# Autodesk Inventor assembly: CL3-100
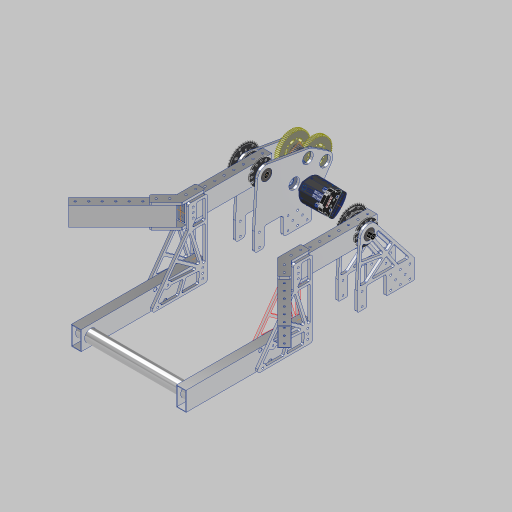
[picture p0: Inventor's stored thumbnail of the model, 512x512]
Saved by Autodesk Inventor 2023.5 (Build 275446000, 446)
## iProperties
Created: 2025-01-28
Part Number: CL3-100
Document SubType Name: Assembly
Designer: slick
Mass: 5966.39 g
Surface Area: 14199.1 cm^2
Volume: 2256.64 cm^3
Density: 2.64392 g/cm^3
Author: slick
## Documents named in this file (25)
- C:\Users\slick\OneDrive\Desktop\2025-ReefScape---CAD\Climber\CL3\CL3-100.iam
- C:\Users\slick\OneDrive\Desktop\2025-ReefScape---CAD\Climber\CL3\CL3-001.ipt
- C:\Users\slick\OneDrive\Desktop\2025-ReefScape---CAD\Climber\CL3\CL3-002.ipt
- C:\Users\slick\OneDrive\Desktop\2025-ReefScape---CAD\Climber\CL3\CL3-003.ipt
- C:\Users\slick\OneDrive\Desktop\2025-ReefScape---CAD\Climber\CL3\CL3-004.ipt
- C:\Users\slick\OneDrive\Desktop\2025-ReefScape---CAD\Climber\CL3\CL3-006.ipt
- C:\Users\slick\OneDrive\Desktop\2025-ReefScape---CAD\Field Items\Full Field\FE-2025\GE-25201.iam
- C:\Users\slick\OneDrive\Desktop\2025-ReefScape---CAD\Climber\CL3\CL3-007.ipt
- C:\Users\slick\OneDrive\Desktop\2025-ReefScape---CAD\Climber\CL3\CL3-009.ipt
- C:\Users\slick\OneDrive\Desktop\2025-ReefScape---CAD\Elevator\EL2\EL2-005.ipt
- C:\Users\slick\OneDrive\Desktop\2025-ReefScape---CAD\Climber\CL3\CL3-010.ipt
- C:\Users\slick\OneDrive\Desktop\2025-ReefScape---CAD\Climber\CL3\CL3-011.ipt
- C:\Users\slick\OneDrive\Desktop\2025-ReefScape---CAD\COMMON PARTS\BEARINGS\0_500_Hex_ID_x_1_125_OD_x_0_313_WD_Flanged_Bearing_v2_217-3875.ipt
- C:\Users\slick\OneDrive\Desktop\2025-ReefScape---CAD\COMMON PARTS\HUBS\WCP-1388.ipt
- C:\Users\slick\OneDrive\Desktop\2025-ReefScape---CAD\COMMON PARTS\SPROCKETS\25\WCP-0967 42t 25_chain.ipt
- C:\Users\slick\OneDrive\Desktop\2025-ReefScape---CAD\Climber\CL3\CL3-012.ipt
- C:\Users\slick\OneDrive\Desktop\2025-ReefScape---CAD\Climber\CL3\CL3-013.ipt
- C:\Users\slick\OneDrive\Desktop\2025-ReefScape---CAD\Climber\CL3\CL3-014.ipt
- C:\Users\slick\OneDrive\Desktop\2025-ReefScape---CAD\Climber\CL3\CL3-015.ipt
- C:\Users\slick\OneDrive\Desktop\2025-ReefScape---CAD\COMMON PARTS\MOTORS\Kracken with Cover and Boards.iam
- C:\Users\slick\OneDrive\Desktop\2025-ReefScape---CAD\COMMON PARTS\GEARS\WCP-1006\WCP-1006.ipt
- C:\Users\slick\OneDrive\Desktop\2025-ReefScape---CAD\COMMON PARTS\GEARS\20dp .5 hex\72t_Aluminum_Spur_Gear_20_DP_1_2_Hex_Bore_217-3576.ipt
- C:\Users\slick\OneDrive\Desktop\2025-ReefScape---CAD\COMMON PARTS\GEARS\20dp .5 hex\66t_Aluminum_Spur_Gear_20_DP_1_2_Hex_Bore_VersaKeys_217-3223.ipt
- C:\Users\slick\OneDrive\Desktop\2025-ReefScape---CAD\COMMON PARTS\GEARS\20dp .5 hex\20t_Aluminum_Spur_Gear_20_DP_1_2_Hex_Bore_217-2702.ipt
- C:\Users\slick\OneDrive\Desktop\2025-ReefScape---CAD\COMMON PARTS\SPROCKETS\25\14t Steel Double Hub Sprocket (#25 Chain, 12 Hex Bore)\14t Steel Double Hub Sprocket (#25 Chain, 12 Hex Bore).ipt
## Components (53 placed, 24 different names)
1. CL3-001:1 — Flush:24, Insert:5, Insert:6, Insert:7, Insert:11, Insert:12, Insert:13, Insert:14, Mate:43, Mate:44, Mate:51, Mate:52, Mate:53, Mate:54, Mate:55, Angle:4, Insert:43, Insert:44
2. CL3-002:1 — Flush:24, Insert:3, Insert:4, Insert:8
3. CL3-003:1 — Insert:26, Insert:27, Mate:56, Mate:57, Insert:48, Insert:49, Insert:50, Insert:51
4. CL3-001:2 — Insert:18, Insert:19, Insert:20, Insert:21, Insert:24, Insert:25, Insert:41, Mate:65, Insert:42, Mate:66, Mate:67
5. CL3-002:2 — Insert:22, Insert:23
6. CL3-003:2 — Mate:29, Flush:26, Flush:27, Mate:33, Mate:34, Insert:15, Insert:16, Insert:17, Insert:45, Insert:46, Insert:47
7. CL3-015:1 — Mate:41, Flush:31, Flush:32, Insert:29, Angle:4, Symmetry:2, Mate:76, Mate:82, Mate:85, Mate:87
8. CL3-004:4 — Insert:39, Mate:68, Flush:33, Symmetry:3
9. CL3-006:1 — Tangent:1, Mate:21, Mate:33, Mate:34, Mate:56, Mate:57
10. GE-25201:1 [sub-assembly] — Mate:20, Tangent:1, Mate:21
11. CL3-007:1 — Mate:29, Flush:26, Flush:27
12. CL3-009:1 — Insert:3, Insert:4, Insert:5, Insert:6
13. CL3-009:2 — Insert:7, Insert:8
14. CL3-013:1 — Insert:43, Insert:44
15. CL3-010:1 — Insert:11, Insert:12, Flush:29
16. CL3-010:2 — Insert:13, Insert:14, Insert:16, Insert:17
17. EL2-005:3 — Insert:15, Insert:45
18. CL3-009:3 — Insert:18, Insert:19
19. CL3-009:4 — Insert:20, Insert:21, Insert:22, Insert:23
20. CL3-010:3 — Insert:25, Flush:29, Flush:30
21. CL3-010:4 — Insert:24, Insert:26, Insert:27, Flush:30
22. CL3-011:1 — Mate:42, Mate:55, Mate:81, Flush:41
23. CL3-015:2 — Mate:41, Flush:31, Flush:32, Insert:28, Symmetry:2, Flush:34, Flush:35, Mate:70, Insert:52, Mate:77, Mate:79, Mate:80, Mate:83
24. 0_500_Hex_ID_x_1_125_OD_x_0_313_WD_Flanged_Bearing_v2_217-3875:1 — Insert:28, Mate:42
25. 0_500_Hex_ID_x_1_125_OD_x_0_313_WD_Flanged_Bearing_v2_217-3875:2 — Insert:29
26. WCP-1388:1 — Mate:43, Mate:44, Mate:51
27. WCP-1388:2 — Mate:52, Mate:53, Mate:54
28. CL3-004:6 — Insert:40, Mate:68, Flush:33, Flush:34, Flush:35, Symmetry:3
29. CL3-011:2 — Mate:64, Mate:67
30. 0_500_Hex_ID_x_1_125_OD_x_0_313_WD_Flanged_Bearing_v2_217-3875:3 — Insert:39
31. 0_500_Hex_ID_x_1_125_OD_x_0_313_WD_Flanged_Bearing_v2_217-3875:4 — Insert:40, Mate:64
32. WCP-1388:3 — Insert:41, Mate:65
33. WCP-1388:4 — Insert:42, Mate:66, Symmetry:4
34. WCP-0967 42t 25_chain:2 — Symmetry:4
35. CL3-012:5
36. CL3-012:6
37. CL3-012:7
38. CL3-012:8
39. CL3-014:1 — Insert:46
40. CL3-014:2 — Insert:47
41. CL3-014:3 — Insert:50
42. CL3-014:4 — Insert:51
43. EL2-005:4 — Insert:48, Insert:49
44. Kracken with Cover and Boards:1 [sub-assembly] — Mate:70, Insert:52, Mate:72, Mate:73, Mate:79
45. WCP-1006:1 — Mate:72, Mate:73
46. 72t_Aluminum_Spur_Gear_20_DP_1_2_Hex_Bore_217-3576:1 — Mate:80, Mate:83, Mate:84
47. 20t_Aluminum_Spur_Gear_20_DP_1_2_Hex_Bore_217-2702:2 — Mate:84, Flush:39, Mate:85
48. 66t_Aluminum_Spur_Gear_20_DP_1_2_Hex_Bore_VersaKeys_217-3223:1 — Mate:76, Flush:39, Mate:86
49. 20t_Aluminum_Spur_Gear_20_DP_1_2_Hex_Bore_217-2702:1 — Mate:77, Flush:38, Mate:86
50. 66t_Aluminum_Spur_Gear_20_DP_1_2_Hex_Bore_VersaKeys_217-3223:2 — Flush:38
51. WCP-0967 42t 25_chain:3 — Insert:53, Insert:54, Mate:82, Flush:40
52. WCP-1388:5 — Insert:53, Insert:54, Mate:81, Flush:41
53. 14t Steel Double Hub Sprocket (#25 Chain, 12 Hex Bore):1 — Mate:87, Flush:40
## Relationships (106: Insert 45, Mate 42, Flush 14, Symmetry 3, Tangent 1, Angle 1)
- Mate:20: GE-25201:1
- Tangent:1: CL3-006:1 ↔ GE-25201:1
- Mate:21 (-76.2 mm): CL3-006:1 ↔ GE-25201:1
- Flush:24: CL3-001:1 ↔ CL3-002:1
- Mate:29: CL3-003:2 ↔ CL3-007:1
- Flush:26: CL3-003:2 ↔ CL3-007:1
- Flush:27: CL3-003:2 ↔ CL3-007:1
- Insert:3: CL3-002:1 ↔ CL3-009:1
- Insert:4: CL3-002:1 ↔ CL3-009:1
- Insert:5: CL3-001:1 ↔ CL3-009:1
- Insert:6: CL3-001:1 ↔ CL3-009:1
- Insert:7: CL3-001:1 ↔ CL3-009:2
- Insert:8: CL3-002:1 ↔ CL3-009:2
- Mate:33: CL3-003:2 ↔ CL3-006:1
- Mate:34: CL3-003:2 ↔ CL3-006:1
- Insert:11: CL3-001:1 ↔ CL3-010:1
- Insert:12: CL3-001:1 ↔ CL3-010:1
- Insert:13: CL3-001:1 ↔ CL3-010:2
- Insert:14: CL3-001:1 ↔ CL3-010:2
- Insert:15: CL3-003:2 ↔ EL2-005:3
- Insert:16: CL3-003:2 ↔ CL3-010:2
- Insert:17: CL3-003:2 ↔ CL3-010:2
- Insert:18: CL3-001:2 ↔ CL3-009:3
- Insert:19: CL3-001:2 ↔ CL3-009:3
- Insert:20: CL3-001:2 ↔ CL3-009:4
- Insert:21: CL3-001:2 ↔ CL3-009:4
- Insert:22: CL3-002:2 ↔ CL3-009:4
- Insert:23: CL3-002:2 ↔ CL3-009:4
- Insert:24: CL3-001:2 ↔ CL3-010:4
- Insert:25: CL3-001:2 ↔ CL3-010:3
- Flush:29: CL3-010:1 ↔ CL3-010:3
- Insert:26: CL3-003:1 ↔ CL3-010:4
- Insert:27: CL3-003:1 ↔ CL3-010:4
- Flush:30: CL3-010:3 ↔ CL3-010:4
- Mate:41 (44.45 mm): CL3-015:1 ↔ CL3-015:2
- Flush:31: CL3-015:1 ↔ CL3-015:2
- Flush:32: CL3-015:1 ↔ CL3-015:2
- Insert:28: CL3-015:2 ↔ 0_500_Hex_ID_x_1_125_OD_x_0_313_WD_Flanged_Bearing_v2_217-3875:1
- Insert:29: CL3-015:1 ↔ 0_500_Hex_ID_x_1_125_OD_x_0_313_WD_Flanged_Bearing_v2_217-3875:2
- Mate:42: CL3-011:1 ↔ 0_500_Hex_ID_x_1_125_OD_x_0_313_WD_Flanged_Bearing_v2_217-3875:1
- Mate:43: CL3-001:1 ↔ WCP-1388:1
- Mate:44: CL3-001:1 ↔ WCP-1388:1
- Mate:51: CL3-001:1 ↔ WCP-1388:1
- Mate:52: CL3-001:1 ↔ WCP-1388:2
- Mate:53: CL3-001:1 ↔ WCP-1388:2
- Mate:54: CL3-001:1 ↔ WCP-1388:2
- Mate:55: CL3-001:1 ↔ CL3-011:1
- Angle:4 (270 deg): CL3-001:1 ↔ CL3-015:1
- Mate:56: CL3-003:1 ↔ CL3-006:1
- Mate:57: CL3-003:1 ↔ CL3-006:1
- Symmetry:2: CL3-015:1 ↔ CL3-015:2
- Mate:59
- [Mate]: CL3-011:2 ↔ 0_500_Hex_ID_x_1_125_OD_x_0_313_WD_Flanged_Bearing_v2_217-3875:3
- [Mate]: WCP-1388:3 ↔ WCP-0967 42t 25_chain:2
- [Mate]: WCP-1388:3 ↔ WCP-0967 42t 25_chain:2
- [Insert]: WCP-0967 42t 25_chain:2 ↔ CL3-012:5
- [Mate]: WCP-1388:3 ↔ CL3-012:5
- [Insert]: WCP-0967 42t 25_chain:2 ↔ CL3-012:6
- [Insert]: WCP-0967 42t 25_chain:2 ↔ CL3-012:8
- [Insert]: WCP-0967 42t 25_chain:2 ↔ CL3-012:7
- Insert:39: CL3-004:4 ↔ 0_500_Hex_ID_x_1_125_OD_x_0_313_WD_Flanged_Bearing_v2_217-3875:3
- Insert:40: CL3-004:6 ↔ 0_500_Hex_ID_x_1_125_OD_x_0_313_WD_Flanged_Bearing_v2_217-3875:4
- Mate:64: CL3-011:2 ↔ 0_500_Hex_ID_x_1_125_OD_x_0_313_WD_Flanged_Bearing_v2_217-3875:4
- Insert:41: CL3-001:2 ↔ WCP-1388:3
- Mate:65: CL3-001:2 ↔ WCP-1388:3
- Insert:42: CL3-001:2 ↔ WCP-1388:4
- Mate:66: CL3-001:2 ↔ WCP-1388:4
- Mate:67: CL3-001:2 ↔ CL3-011:2
- Mate:68 (44.45 mm): CL3-004:4 ↔ CL3-004:6
- Flush:33: CL3-004:4 ↔ CL3-004:6
- Flush:34: CL3-015:2 ↔ CL3-004:6
- Flush:35: CL3-015:2 ↔ CL3-004:6
- Symmetry:3: CL3-004:4 ↔ CL3-004:6
- Symmetry:4: WCP-1388:4 ↔ WCP-0967 42t 25_chain:2
- Mate:69
- Insert:43: CL3-001:1 ↔ CL3-013:1
- Insert:44: CL3-001:1 ↔ CL3-013:1
- Insert:45: CL3-003:2 ↔ EL2-005:3
- Insert:46: CL3-003:2 ↔ CL3-014:1
- Insert:47: CL3-003:2 ↔ CL3-014:2
- Insert:48: CL3-003:1 ↔ EL2-005:4
- Insert:49: CL3-003:1 ↔ EL2-005:4
- Insert:50: CL3-003:1 ↔ CL3-014:3
- Insert:51: CL3-003:1 ↔ CL3-014:4
- Mate:70: CL3-015:2 ↔ Kracken with Cover and Boards:1
- Insert:52: CL3-015:2 ↔ Kracken with Cover and Boards:1
- Mate:72: Kracken with Cover and Boards:1 ↔ WCP-1006:1
- Mate:73 (3.175 mm): Kracken with Cover and Boards:1 ↔ WCP-1006:1
- Mate:76: CL3-015:1 ↔ 66t_Aluminum_Spur_Gear_20_DP_1_2_Hex_Bore_VersaKeys_217-3223:1
- Mate:77: CL3-015:2 ↔ 20t_Aluminum_Spur_Gear_20_DP_1_2_Hex_Bore_217-2702:1
- [Mate]: CL3-015:2 ↔ 66t_Aluminum_Spur_Gear_20_DP_1_2_Hex_Bore_VersaKeys_217-3223:2
- Mate:79: CL3-015:2 ↔ Kracken with Cover and Boards:1
- Mate:80: CL3-015:2 ↔ 72t_Aluminum_Spur_Gear_20_DP_1_2_Hex_Bore_217-3576:1
- Flush:38: 20t_Aluminum_Spur_Gear_20_DP_1_2_Hex_Bore_217-2702:1 ↔ 66t_Aluminum_Spur_Gear_20_DP_1_2_Hex_Bore_VersaKeys_217-3223:2
- Insert:53: WCP-0967 42t 25_chain:3 ↔ WCP-1388:5
- Insert:54: WCP-0967 42t 25_chain:3 ↔ WCP-1388:5
- Mate:81: CL3-011:1 ↔ WCP-1388:5
- Mate:82 (3.175 mm): CL3-015:1 ↔ WCP-0967 42t 25_chain:3
- Mate:83 (3.175 mm): CL3-015:2 ↔ 72t_Aluminum_Spur_Gear_20_DP_1_2_Hex_Bore_217-3576:1
- Mate:84: 72t_Aluminum_Spur_Gear_20_DP_1_2_Hex_Bore_217-3576:1 ↔ 20t_Aluminum_Spur_Gear_20_DP_1_2_Hex_Bore_217-2702:2
- Flush:39: 20t_Aluminum_Spur_Gear_20_DP_1_2_Hex_Bore_217-2702:2 ↔ 66t_Aluminum_Spur_Gear_20_DP_1_2_Hex_Bore_VersaKeys_217-3223:1
- Mate:85 (3.175 mm): CL3-015:1 ↔ 20t_Aluminum_Spur_Gear_20_DP_1_2_Hex_Bore_217-2702:2
- Mate:86: 66t_Aluminum_Spur_Gear_20_DP_1_2_Hex_Bore_VersaKeys_217-3223:1 ↔ 20t_Aluminum_Spur_Gear_20_DP_1_2_Hex_Bore_217-2702:1
- Mate:87: CL3-015:1 ↔ 14t Steel Double Hub Sprocket (#25 Chain, 12 Hex Bore):1
- Flush:40: WCP-0967 42t 25_chain:3 ↔ 14t Steel Double Hub Sprocket (#25 Chain, 12 Hex Bore):1
- Flush:41: CL3-011:1 ↔ WCP-1388:5
## Named parameters: d209_d182 = 0 mm, d210_d190 = 0 mm, d211_d191 = 0 mm, d212_d202 = 0 mm, d213_d203 = 0 mm, d214_d204 = 0 mm, d215_d205 = 0 mm, d216_d206 = 0 mm
